# Autodesk Inventor assembly: AlberoMontato
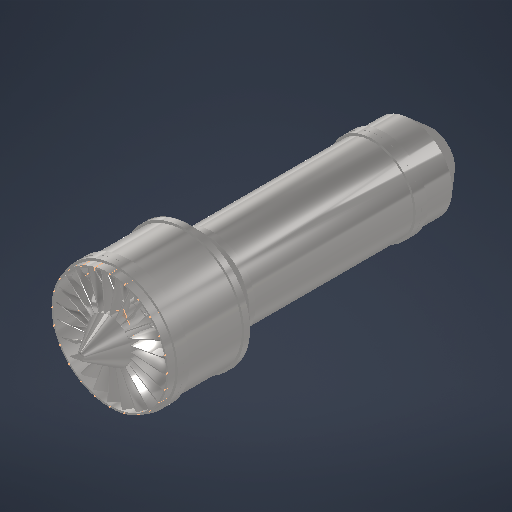
[picture p0: Inventor's stored thumbnail of the model, 512x512]
Saved by Autodesk Inventor 2026.2 (Build 302298010, 298A)
## iProperties
Created: 2026-04-26
Part Number: AlberoMontato
Document SubType Name: Assembly
Designer: Yan
Author: Yan
## Documents named in this file (13)
- C:\Users\Yan\Desktop\Turbina\AlberoMontato.iam
- C:\Users\Yan\Desktop\Turbina\Albero Cavo.ipt
- C:\Users\Yan\Desktop\Turbina\HPC.iam
- C:\Users\Yan\Desktop\Turbina\LPC.iam
- C:\Users\Yan\Documents\Inventor\Content Center Files\R2026\en-US\DIN 5412 - T1  NU\DIN 5412 T1 - NU1020 - 100 x 150 x 24.ipt
- C:\Users\Yan\Desktop\Turbina\HPC+LPC.iam
- C:\Users\Yan\Desktop\Turbina\SFD_CuscinettoRadiale180x150x0.20.ipt
- C:\Users\Yan\Desktop\Turbina\Corpo2-3.iam
- C:\Users\Yan\Desktop\Turbina\Corpo1.iam
- C:\Users\Yan\Desktop\Turbina\CorpoInternoTurbinaAssemblato.iam
- C:\Users\Yan\Desktop\Turbina\Collegamento2.ipt
- C:\Users\Yan\Desktop\Turbina\ConoDiffusione.ipt
- C:\Users\Yan\Desktop\Turbina\ConoEntrata.ipt
## Components (17 placed, 12 different names)
1. Albero Cavo:1 — Mate:1, Mate:2, Mate:3, Flush:1, Mate:4, Mate:6, Mate:8, Mate:9, Mate:12, Mate:15, Mate:16, Mate:18, Mate:20, Mate:21, Mate:22, Mate:23, Mate:25, Mate:26, Mate:27, Mate:30
2. HPC:1 [sub-assembly] — Mate:1, Mate:3, Mate:5, Mate:13
3. LPC:1 [sub-assembly] — Mate:2, Flush:1, Mate:7
4. DIN 5412 - T1 NU NU1020 - 100 x 150 x 24:1 — Mate:4, Mate:5
5. DIN 5412 - T1 NU NU1020 - 100 x 150 x 24:2 — Mate:6, Mate:7, Flush:3
6. HPC+LPC:1 [sub-assembly] — Mate:8, Mate:9, Mate:19
7. SFD_CuscinettoRadiale180x150x0.20:1 — Mate:12, Mate:13, Flush:7
8. SFD_CuscinettoRadiale180x150x0.20:3 — Mate:15, Flush:3, Flush:6
9. DIN 5412 - T1 NU NU1020 - 100 x 150 x 24:3 — Mate:16, Flush:4, Mate:19
10. SFD_CuscinettoRadiale180x150x0.20:4 — Mate:18, Flush:4, Flush:5, Mate:29
11. Corpo2-3:1 [sub-assembly] — Mate:20, Flush:5
12. Corpo2-3:2 [sub-assembly] — Mate:21, Flush:6
13. Corpo1:1 [sub-assembly] — Mate:22, Flush:7, Mate:24, Mate:28
14. CorpoInternoTurbinaAssemblato:1 [sub-assembly] — Mate:23, Mate:24
15. Collegamento2:1 — Mate:25, Mate:29
16. ConoDiffusione:1 — Mate:26, Mate:27
17. ConoEntrata:1 — Mate:28, Mate:30
## Relationships (32: Mate 26, Flush 6)
- Mate:1: Albero Cavo:1 ↔ HPC:1
- Mate:2: Albero Cavo:1 ↔ LPC:1
- Mate:3: Albero Cavo:1 ↔ HPC:1
- Flush:1: Albero Cavo:1 ↔ LPC:1
- Mate:4: Albero Cavo:1 ↔ DIN 5412 - T1 NU NU1020 - 100 x 150 x 24:1
- Mate:5: HPC:1 ↔ DIN 5412 - T1 NU NU1020 - 100 x 150 x 24:1
- Mate:6: Albero Cavo:1 ↔ DIN 5412 - T1 NU NU1020 - 100 x 150 x 24:2
- Mate:7: LPC:1 ↔ DIN 5412 - T1 NU NU1020 - 100 x 150 x 24:2
- Mate:8: Albero Cavo:1 ↔ HPC+LPC:1
- Mate:9: Albero Cavo:1 ↔ HPC+LPC:1
- Mate:12: Albero Cavo:1 ↔ SFD_CuscinettoRadiale180x150x0.20:1
- Mate:13: HPC:1 ↔ SFD_CuscinettoRadiale180x150x0.20:1
- Mate:15: Albero Cavo:1 ↔ SFD_CuscinettoRadiale180x150x0.20:3
- Flush:3: DIN 5412 - T1 NU NU1020 - 100 x 150 x 24:2 ↔ SFD_CuscinettoRadiale180x150x0.20:3
- Mate:16: Albero Cavo:1 ↔ DIN 5412 - T1 NU NU1020 - 100 x 150 x 24:3
- Mate:18: Albero Cavo:1 ↔ SFD_CuscinettoRadiale180x150x0.20:4
- Flush:4: DIN 5412 - T1 NU NU1020 - 100 x 150 x 24:3 ↔ SFD_CuscinettoRadiale180x150x0.20:4
- Mate:19: HPC+LPC:1 ↔ DIN 5412 - T1 NU NU1020 - 100 x 150 x 24:3
- Mate:20: Albero Cavo:1 ↔ Corpo2-3:1
- Flush:5: SFD_CuscinettoRadiale180x150x0.20:4 ↔ Corpo2-3:1
- Mate:21: Albero Cavo:1 ↔ Corpo2-3:2
- Flush:6: SFD_CuscinettoRadiale180x150x0.20:3 ↔ Corpo2-3:2
- Mate:22: Albero Cavo:1 ↔ Corpo1:1
- Flush:7: SFD_CuscinettoRadiale180x150x0.20:1 ↔ Corpo1:1
- Mate:23: Albero Cavo:1 ↔ CorpoInternoTurbinaAssemblato:1
- Mate:24: Corpo1:1 ↔ CorpoInternoTurbinaAssemblato:1
- Mate:25: Albero Cavo:1 ↔ Collegamento2:1
- Mate:26: Albero Cavo:1 ↔ ConoDiffusione:1
- Mate:27: Albero Cavo:1 ↔ ConoDiffusione:1
- Mate:28: Corpo1:1 ↔ ConoEntrata:1
- Mate:29: SFD_CuscinettoRadiale180x150x0.20:4 ↔ Collegamento2:1
- Mate:30: Albero Cavo:1 ↔ ConoEntrata:1
